# Autodesk Inventor assembly: Terminalblock
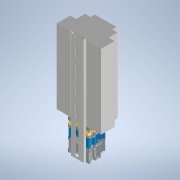
[picture p0: Inventor's stored thumbnail of the model, 180x180]
Saved by Autodesk Inventor 2020 (Build 240168000, 168)
## iProperties
Created: 2019-12-11
Part Number: Terminalblock
Document SubType Name: Assembly
Designer: nicoc
Author: nicoc
## Documents named in this file (8)
- D:\Repos\P5-AIonFPGA\cad\Case\Terminalblock\Terminalblock.iam
- D:\Repos\P5-AIonFPGA\cad\Case\DinRail223mm.ipt
- D:\Repos\P5-AIonFPGA\cad\Case\Supply.ipt
- D:\Repos\P5-AIonFPGA\cad\Case\Terminalblock\TerminalBlockBlue\TerminalBlockBlue.iam
- D:\Repos\P5-AIonFPGA\cad\Case\Terminalblock\TerminalBlockGreen\TerminalBlockGreen.iam
- D:\Repos\P5-AIonFPGA\cad\Case\Terminalblock\TerminalBlockGrey\TerminalBlockGrey.iam
- D:\Repos\P5-AIonFPGA\cad\Case\Terminalblock\EndCover\EndCover.iam
- D:\Repos\P5-AIonFPGA\cad\Case\Terminalblock\EndClamp\EndClamp.iam
## Components (17 placed, 7 different names)
1. DinRail223mm:1 — Flush:1, Mate:1, Mate:2, Mate:11, Mate:12, Mate:14, Mate:16, Mate:17, Mate:19, Mate:20, Mate:24, Mate:26, Mate:28, Mate:29
2. Supply:1 — Flush:1, Mate:1, Mate:2, Flush:2, Mate:3, Flush:3
3. Supply:2 — Flush:2, Mate:3, Flush:3, Mate:10
4. TerminalBlockBlue:1 [sub-assembly] — Flush:4, Mate:4, Flush:5, Mate:16, Mate:17, Mate:18
5. TerminalBlockBlue:2 [sub-assembly] — Flush:4, Mate:4, Flush:5, Flush:6, Flush:7, Mate:5
6. TerminalBlockBlue:3 [sub-assembly] — Flush:6, Flush:7, Mate:5, Mate:6, Flush:8, Flush:9
7. TerminalBlockGreen:1 [sub-assembly] — Mate:8, Flush:12, Flush:13, Flush:15, Mate:13, Flush:16
8. TerminalBlockGrey:1 [sub-assembly] — Mate:21, Flush:17, Flush:18, Flush:19, Flush:20, Mate:22
9. TerminalBlockGrey:2 [sub-assembly] — Flush:19, Flush:20, Mate:22, Flush:22, Mate:26, Mate:27
10. TerminalBlockGrey:3 [sub-assembly] — Mate:21, Flush:17, Flush:18, Flush:21, Mate:23, Mate:24
11. EndCover:1 [sub-assembly] — Flush:21, Flush:22, Mate:23, Mate:25
12. EndCover:2 [sub-assembly] — Mate:6, Flush:8, Flush:9, Mate:15
13. EndCover:3 [sub-assembly] — Mate:8, Flush:12, Flush:13, Mate:9, Flush:14
14. EndClamp:1 [sub-assembly] — Mate:27, Mate:28, Mate:29
15. EndClamp:2 [sub-assembly] — Mate:13, Flush:16, Mate:14, Mate:15
16. EndClamp:3 [sub-assembly] — Mate:9, Flush:14, Flush:15, Mate:10, Mate:11, Mate:12
17. EndClamp:4 [sub-assembly] — Mate:18, Mate:19, Mate:20, Mate:25
## Relationships (48: Mate 28, Flush 20)
- Flush:1 (1.875 mm): DinRail223mm:1 ↔ Supply:1
- Mate:1: DinRail223mm:1 ↔ Supply:1
- Mate:2: DinRail223mm:1 ↔ Supply:1
- Flush:2: Supply:1 ↔ Supply:2
- Mate:3: Supply:1 ↔ Supply:2
- Flush:3: Supply:1 ↔ Supply:2
- Flush:4: TerminalBlockBlue:1 ↔ TerminalBlockBlue:2
- Mate:4: TerminalBlockBlue:1 ↔ TerminalBlockBlue:2
- Flush:5: TerminalBlockBlue:1 ↔ TerminalBlockBlue:2
- Flush:6: TerminalBlockBlue:2 ↔ TerminalBlockBlue:3
- Flush:7: TerminalBlockBlue:2 ↔ TerminalBlockBlue:3
- Mate:5: TerminalBlockBlue:2 ↔ TerminalBlockBlue:3
- Mate:6: TerminalBlockBlue:3 ↔ EndCover:2
- Flush:8: TerminalBlockBlue:3 ↔ EndCover:2
- Flush:9: TerminalBlockBlue:3 ↔ EndCover:2
- Mate:8: TerminalBlockGreen:1 ↔ EndCover:3
- Flush:12: TerminalBlockGreen:1 ↔ EndCover:3
- Flush:13: TerminalBlockGreen:1 ↔ EndCover:3
- Mate:9: EndCover:3 ↔ EndClamp:3
- Flush:14: EndCover:3 ↔ EndClamp:3
- Flush:15: TerminalBlockGreen:1 ↔ EndClamp:3
- Mate:10: Supply:2 ↔ EndClamp:3
- Mate:11: DinRail223mm:1 ↔ EndClamp:3
- Mate:12: DinRail223mm:1 ↔ EndClamp:3
- Mate:13: TerminalBlockGreen:1 ↔ EndClamp:2
- Flush:16: TerminalBlockGreen:1 ↔ EndClamp:2
- Mate:14: DinRail223mm:1 ↔ EndClamp:2
- Mate:15: EndCover:2 ↔ EndClamp:2
- Mate:16: DinRail223mm:1 ↔ TerminalBlockBlue:1
- Mate:17: DinRail223mm:1 ↔ TerminalBlockBlue:1
- Mate:18: TerminalBlockBlue:1 ↔ EndClamp:4
- Mate:19: DinRail223mm:1 ↔ EndClamp:4
- Mate:20: DinRail223mm:1 ↔ EndClamp:4
- Mate:21: TerminalBlockGrey:1 ↔ TerminalBlockGrey:3
- Flush:17: TerminalBlockGrey:1 ↔ TerminalBlockGrey:3
- Flush:18: TerminalBlockGrey:1 ↔ TerminalBlockGrey:3
- Flush:19: TerminalBlockGrey:1 ↔ TerminalBlockGrey:2
- Flush:20: TerminalBlockGrey:1 ↔ TerminalBlockGrey:2
- Mate:22: TerminalBlockGrey:1 ↔ TerminalBlockGrey:2
- Flush:21: TerminalBlockGrey:3 ↔ EndCover:1
- Flush:22: TerminalBlockGrey:2 ↔ EndCover:1
- Mate:23: TerminalBlockGrey:3 ↔ EndCover:1
- Mate:24: DinRail223mm:1 ↔ TerminalBlockGrey:3
- Mate:25: EndCover:1 ↔ EndClamp:4
- Mate:26: DinRail223mm:1 ↔ TerminalBlockGrey:2
- Mate:27: TerminalBlockGrey:2 ↔ EndClamp:1
- Mate:28: DinRail223mm:1 ↔ EndClamp:1
- Mate:29: DinRail223mm:1 ↔ EndClamp:1
